# Autodesk Inventor assembly: ASSEMBLY FOR STORAGE SYSTEM
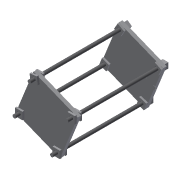
[picture p0: Inventor's stored thumbnail of the model, 180x180]
Saved by Autodesk Inventor 2019 (Build 230136000, 136)
## iProperties
Created: 2019-10-14
Part Number: ASSEMBLY FOR STORAGE SYSTEM
Document SubType Name: Assembly
Designer: Admin
Author: Admin
## Documents named in this file (5)
- C:\Users\Admin\Documents\ASSEMBLY FOR STORAGE SYSTEM.iam
- C:\Users\Admin\Documents\STAND PLATE FOR STORSGE SYSTEM.ipt
- C:\Users\Admin\Documents\small nu 1.ipt
- C:\Users\Admin\Documents\nut for capping system.ipt
- C:\Users\Admin\Documents\ir sensor.ipt
## Components (19 placed, 4 different names)
1. STAND PLATE FOR STORSGE SYSTEM:1 — Mate:3, Mate:4, Mate:5, Mate:6, Mate:7, Mate:8, Mate:9, Mate:10, Mate:11, Mate:16, Mate:17, Mate:18, Mate:19, Rotational:1
2. small nu 1:1 — Mate:4, Mate:5, Mate:13, Mate:20, Mate:24, Mate:32
3. small nu 1:2 — Mate:7, Mate:9, Mate:12, Mate:21, Mate:26, Mate:35
4. small nu 1:3 — Mate:6, Mate:10, Mate:15, Mate:23, Mate:25, Mate:34
5. small nu 1:4 — Mate:8, Mate:11, Mate:14, Mate:22, Mate:27, Mate:33
6. nut for capping system:1 — Mate:12, Mate:19
7. nut for capping system:2 — Mate:13, Mate:17
8. nut for capping system:3 — Mate:14, Mate:18
9. nut for capping system:4 — Mate:15, Mate:16
10. nut for capping system:5 — Mate:20, Mate:31
11. nut for capping system:6 — Mate:22, Mate:30
12. nut for capping system:7 — Mate:21, Mate:29
13. nut for capping system:8 — Mate:23, Mate:28
14. STAND PLATE FOR STORSGE SYSTEM:2 — Mate:24, Mate:25, Mate:26, Mate:27, Mate:28, Mate:29, Mate:30, Mate:31, Mate:36, Mate:37, Mate:38, Mate:39
15. nut for capping system:9 — Mate:32, Mate:36
16. nut for capping system:10 — Mate:33, Mate:38
17. nut for capping system:11 — Mate:34, Mate:37
18. nut for capping system:12 — Mate:35, Mate:39
19. ir sensor:1 — Rotational:1
## Relationships (38: Mate 37, RevoluteJoint 1)
- Mate:3: STAND PLATE FOR STORSGE SYSTEM:1
- Mate:4: STAND PLATE FOR STORSGE SYSTEM:1 ↔ small nu 1:1
- Mate:5: STAND PLATE FOR STORSGE SYSTEM:1 ↔ small nu 1:1
- Mate:6: STAND PLATE FOR STORSGE SYSTEM:1 ↔ small nu 1:3
- Mate:7: STAND PLATE FOR STORSGE SYSTEM:1 ↔ small nu 1:2
- Mate:8: STAND PLATE FOR STORSGE SYSTEM:1 ↔ small nu 1:4
- Mate:9: STAND PLATE FOR STORSGE SYSTEM:1 ↔ small nu 1:2
- Mate:10: STAND PLATE FOR STORSGE SYSTEM:1 ↔ small nu 1:3
- Mate:11: STAND PLATE FOR STORSGE SYSTEM:1 ↔ small nu 1:4
- Mate:12: small nu 1:2 ↔ nut for capping system:1
- Mate:13: small nu 1:1 ↔ nut for capping system:2
- Mate:14: small nu 1:4 ↔ nut for capping system:3
- Mate:15: small nu 1:3 ↔ nut for capping system:4
- Mate:16: STAND PLATE FOR STORSGE SYSTEM:1 ↔ nut for capping system:4
- Mate:17: STAND PLATE FOR STORSGE SYSTEM:1 ↔ nut for capping system:2
- Mate:18: STAND PLATE FOR STORSGE SYSTEM:1 ↔ nut for capping system:3
- Mate:19: STAND PLATE FOR STORSGE SYSTEM:1 ↔ nut for capping system:1
- Mate:20: small nu 1:1 ↔ nut for capping system:5
- Mate:21: small nu 1:2 ↔ nut for capping system:7
- Mate:22: small nu 1:4 ↔ nut for capping system:6
- Mate:23: small nu 1:3 ↔ nut for capping system:8
- Mate:24: small nu 1:1 ↔ STAND PLATE FOR STORSGE SYSTEM:2
- Mate:25: small nu 1:3 ↔ STAND PLATE FOR STORSGE SYSTEM:2
- Mate:26: small nu 1:2 ↔ STAND PLATE FOR STORSGE SYSTEM:2
- Mate:27: small nu 1:4 ↔ STAND PLATE FOR STORSGE SYSTEM:2
- Mate:28: nut for capping system:8 ↔ STAND PLATE FOR STORSGE SYSTEM:2
- Mate:29: nut for capping system:7 ↔ STAND PLATE FOR STORSGE SYSTEM:2
- Mate:30: nut for capping system:6 ↔ STAND PLATE FOR STORSGE SYSTEM:2
- Mate:31: nut for capping system:5 ↔ STAND PLATE FOR STORSGE SYSTEM:2
- Mate:32: small nu 1:1 ↔ nut for capping system:9
- Mate:33: small nu 1:4 ↔ nut for capping system:10
- Mate:34: small nu 1:3 ↔ nut for capping system:11
- Mate:35: small nu 1:2 ↔ nut for capping system:12
- Mate:36: STAND PLATE FOR STORSGE SYSTEM:2 ↔ nut for capping system:9
- Mate:37: STAND PLATE FOR STORSGE SYSTEM:2 ↔ nut for capping system:11
- Mate:38: STAND PLATE FOR STORSGE SYSTEM:2 ↔ nut for capping system:10
- Mate:39: STAND PLATE FOR STORSGE SYSTEM:2 ↔ nut for capping system:12
- Rotational:1 [RevoluteJoint]: STAND PLATE FOR STORSGE SYSTEM:1 ↔ ir sensor:1
